# Autodesk Inventor assembly: Door Levered [B]
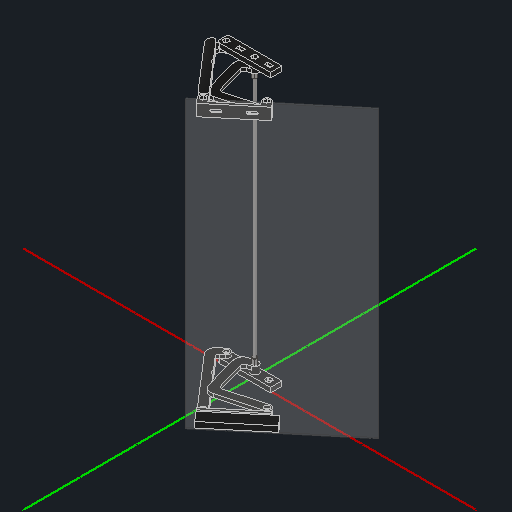
[picture p0: Inventor's stored thumbnail of the model, 512x512]
Saved by Autodesk Inventor 2022.2 (Build 262287010, 287A)
## iProperties
Created: 2022-03-16
Part Number: Door Levered [B]
Document SubType Name: Assembly
Designer: sleib
Author: sleib
## Documents named in this file (11)
- C:\Users\sleib\Projekte\Voron-2\CAD\Inventor\Door Levered [B].iam
- C:\Users\sleib\Projekte\Voron-2\CAD\Inventor\Door Basis.ipt
- C:\Users\sleib\Projekte\Voron-2\CAD\Inventor\Door Handle.ipt
- C:\Users\sleib\Projekte\Voron-2\CAD\Inventor\Door Lever [B].ipt
- C:\Users\sleib\Projekte\Voron-2\CAD\Inventor\Door Lever2 [B].ipt
- C:\Users\sleib\Projekte\Voron-2\CAD\Inventor\Door Panel [B].ipt
- C:\Users\sleib\Projekte\Voron-2\CAD\Inventor\Door Lever [A].ipt
- C:\Users\sleib\Projekte\Voron-2\CAD\Inventor\Door Lever2 [A].ipt
- C:\Users\sleib\Projekte\Voron-2\CAD\Inventor\Door Panel [A].ipt
- C:\Users\sleib\Projekte\Voron-2\CAD\Inventor\Panel Door.ipt
- C:\Users\sleib\Projekte\Voron-2\CAD\Inventor\Door Axis.ipt
## Components (11 placed, 10 different names)
1. Door Basis:1 — Passend:1, Passend:2, Passend:3, Passend:4, Fluchtend:1, Fluchtend:2, Passend:17, Fluchtend:6
2. Door Handle:1 — Fluchtend:4, Passend:20, Fluchtend:5
3. Door Lever [B]:1 — Passend:1, Passend:4, Passend:5, Passend:8
4. Door Lever2 [B]:1 — Passend:2, Passend:3, Passend:6, Passend:7, Passend:21, Passend:24, Passend:25
5. Door Panel [B]:1 — Passend:5, Passend:6, Passend:7, Passend:8, Passend:18, Fluchtend:3, Symmetrie:1, Fluchtend:4, Fluchtend:5, Fluchtend:6
6. Door Basis:2 — Passend:9, Passend:10, Passend:11, Passend:12, Fluchtend:1, Fluchtend:2, Passend:17
7. Door Lever [A]:1 — Passend:9, Passend:11, Passend:13, Passend:15
8. Door Lever2 [A]:1 — Passend:10, Passend:12, Passend:14, Passend:16, Passend:22, Passend:23
9. Door Panel [A]:1 — Passend:13, Passend:14, Passend:15, Passend:16, Passend:19, Symmetrie:1
10. Panel Door:1 — Passend:18, Passend:19, Fluchtend:3, Passend:20
11. Door Axis:1 — Passend:21, Passend:22, Passend:23, Passend:24, Passend:25
## Relationships (32: Mate 25, Flush 6, Symmetry 1)
- Passend:1 [Mate]: Door Basis:1 ↔ Door Lever [B]:1
- Passend:2 [Mate]: Door Basis:1 ↔ Door Lever2 [B]:1
- Passend:3 [Mate]: Door Basis:1 ↔ Door Lever2 [B]:1
- Passend:4 [Mate]: Door Basis:1 ↔ Door Lever [B]:1
- Passend:5 [Mate]: Door Lever [B]:1 ↔ Door Panel [B]:1
- Passend:6 [Mate]: Door Lever2 [B]:1 ↔ Door Panel [B]:1
- Passend:7 [Mate]: Door Lever2 [B]:1 ↔ Door Panel [B]:1
- Passend:8 [Mate]: Door Lever [B]:1 ↔ Door Panel [B]:1
- Passend:9 [Mate]: Door Basis:2 ↔ Door Lever [A]:1
- Passend:10 [Mate]: Door Basis:2 ↔ Door Lever2 [A]:1
- Passend:11 [Mate]: Door Basis:2 ↔ Door Lever [A]:1
- Passend:12 [Mate]: Door Basis:2 ↔ Door Lever2 [A]:1
- Passend:13 [Mate]: Door Lever [A]:1 ↔ Door Panel [A]:1
- Passend:14 [Mate]: Door Lever2 [A]:1 ↔ Door Panel [A]:1
- Passend:15 [Mate]: Door Lever [A]:1 ↔ Door Panel [A]:1
- Passend:16 [Mate]: Door Lever2 [A]:1 ↔ Door Panel [A]:1
- Fluchtend:1 [Flush]: Door Basis:1 ↔ Door Basis:2
- Fluchtend:2 [Flush]: Door Basis:1 ↔ Door Basis:2
- Passend:17 [Mate] (-490 mm): Door Basis:1 ↔ Door Basis:2
- Passend:18 [Mate]: Door Panel [B]:1 ↔ Panel Door:1
- Passend:19 [Mate]: Door Panel [A]:1 ↔ Panel Door:1
- Fluchtend:3 [Flush] (13.4 mm): Door Panel [B]:1 ↔ Panel Door:1
- Symmetrie:1: Door Panel [B]:1 ↔ Door Panel [A]:1
- Fluchtend:4 [Flush]: Door Handle:1 ↔ Door Panel [B]:1
- Passend:20 [Mate]: Door Handle:1 ↔ Panel Door:1
- Fluchtend:5 [Flush]: Door Handle:1 ↔ Door Panel [B]:1
- Fluchtend:6 [Flush] (3 mm): Door Basis:1 ↔ Door Panel [B]:1
- Passend:21 [Mate]: Door Lever2 [B]:1 ↔ Door Axis:1
- Passend:22 [Mate]: Door Lever2 [A]:1 ↔ Door Axis:1
- Passend:23 [Mate]: Door Lever2 [A]:1 ↔ Door Axis:1
- Passend:24 [Mate]: Door Lever2 [B]:1 ↔ Door Axis:1
- Passend:25 [Mate]: Door Lever2 [B]:1 ↔ Door Axis:1
